# Autodesk Inventor assembly: Assembly2
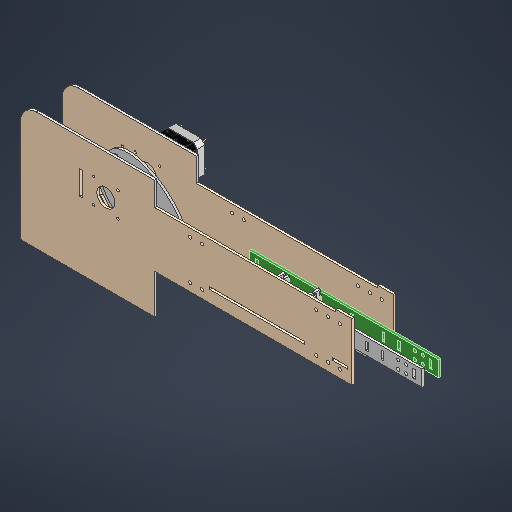
[picture p0: Inventor's stored thumbnail of the model, 512x512]
Saved by Autodesk Inventor 2027 (Build 310192000, 192)
## iProperties
Created: 2026-05-09
Part Number: Assembly2
Document SubType Name: Assembly
Designer: alexy
Author: alexy
## Documents named in this file (9)
- C:\Users\alexy\OneDrive\文件\Carinventor\1stmodel\Assembly2.iam
- C:\Users\alexy\OneDrive\文件\Carinventor\1stmodel\Nema 17 stepper motor.ipt
- C:\Users\alexy\OneDrive\文件\Carinventor\1stmodel\Frontrail.ipt
- C:\Users\alexy\OneDrive\文件\Carinventor\1stmodel\Moving_rail.ipt
- C:\Users\alexy\OneDrive\文件\Carinventor\1stmodel\Middle_bar.ipt
- C:\Users\alexy\OneDrive\文件\Carinventor\1stmodel\Spring_holder.ipt
- C:\Users\alexy\OneDrive\文件\Carinventor\1stmodel\Spring_holder2.ipt
- C:\Users\alexy\OneDrive\文件\Carinventor\1stmodel\Rail1st_withD.ipt
- C:\Users\alexy\OneDrive\文件\Carinventor\1stmodel\Sideboard2.ipt
## Components (11 placed, 8 different names)
1. Nema 17 stepper motor:1 — Insert:2, Angle:1, Mate:23, Angle:3, Mate:24
2. Frontrail:1 — Mate:25, Mate:27, Mate:28
3. Moving_rail:1 — Mate:9, Mate:10, Mate:11, Mate:12, Mate:13, Mate:14, Mate:29, Mate:31
4. Middle_bar:1 — Mate:9, Mate:10, Mate:11, Mate:17, Mate:18, Mate:19, Mate:20, Mate:21, Mate:22, Mate:30
5. Middle_bar:2 — Mate:12, Mate:13, Mate:14
6. Spring_holder:1 — Mate:17, Mate:18, Mate:19
7. Spring_holder2:1 — Mate:20, Mate:21, Mate:22
8. Rail1st_withD:1 — Insert:2, Angle:1, Angle:2, Insert:3
9. Rail1st_withD:2 — Angle:2, Insert:3
10. Sideboard2:1 — Mate:23, Angle:3, Mate:24, Mate:25, Mate:27, Mate:28, Mate:29, Mate:30, Mate:31, Flush:1, Flush:2, Mate:32
11. Sideboard2:2 — Flush:1, Flush:2, Mate:32
## Relationships (28: Mate 21, Angle 3, Insert 2, Flush 2)
- Mate:9: Moving_rail:1 ↔ Middle_bar:1
- Mate:10: Moving_rail:1 ↔ Middle_bar:1
- Mate:11: Moving_rail:1 ↔ Middle_bar:1
- Mate:12: Moving_rail:1 ↔ Middle_bar:2
- Mate:13: Moving_rail:1 ↔ Middle_bar:2
- Mate:14: Moving_rail:1 ↔ Middle_bar:2
- Mate:17: Middle_bar:1 ↔ Spring_holder:1
- Mate:18: Middle_bar:1 ↔ Spring_holder:1
- Mate:19: Middle_bar:1 ↔ Spring_holder:1
- Mate:20: Middle_bar:1 ↔ Spring_holder2:1
- Mate:21: Middle_bar:1 ↔ Spring_holder2:1
- Mate:22: Middle_bar:1 ↔ Spring_holder2:1
- Insert:2 (19 mm): Nema 17 stepper motor:1 ↔ Rail1st_withD:1
- Angle:1 (3381 deg): Nema 17 stepper motor:1 ↔ Rail1st_withD:1
- Angle:2 (0 deg): Rail1st_withD:1 ↔ Rail1st_withD:2
- Insert:3 (15 mm): Rail1st_withD:1 ↔ Rail1st_withD:2
- Mate:23: Nema 17 stepper motor:1 ↔ Sideboard2:1
- Angle:3 (180 deg): Nema 17 stepper motor:1 ↔ Sideboard2:1
- Mate:24: Nema 17 stepper motor:1 ↔ Sideboard2:1
- Mate:25: Frontrail:1 ↔ Sideboard2:1
- Mate:27: Frontrail:1 ↔ Sideboard2:1
- Mate:28: Frontrail:1 ↔ Sideboard2:1
- Mate:29: Moving_rail:1 ↔ Sideboard2:1
- Mate:30 (5 mm): Middle_bar:1 ↔ Sideboard2:1
- Mate:31 (10 mm): Moving_rail:1 ↔ Sideboard2:1
- Flush:1: Sideboard2:1 ↔ Sideboard2:2
- Flush:2: Sideboard2:1 ↔ Sideboard2:2
- Mate:32 (50 mm): Sideboard2:1 ↔ Sideboard2:2
